# Autodesk Inventor assembly: Carrier
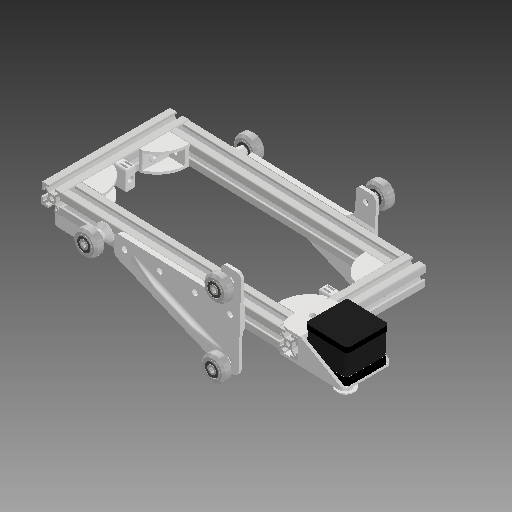
[picture p0: Inventor's stored thumbnail of the model, 512x512]
Saved by Autodesk Inventor 2020 (Build 240168000, 168)
## iProperties
Created: 2020-10-19
Part Number: Carrier
Document SubType Name: Assembly
Designer: DDeGo
Author: DDeGo
## Documents named in this file (13)
- C:\Users\DDeGo\Documents\Drew\Projects\De-Cruster\cad\Carrier.iam
- C:\Users\DDeGo\Documents\Drew\Projects\De-Cruster\cad\Cart Carrier.ipt
- C:\Users\DDeGo\Documents\Drew\Projects\De-Cruster\cad\VWheel.iam
- C:\Users\DDeGo\Documents\Drew\Projects\De-Cruster\cad\2020 Extrusion 200mm.ipt
- C:\Users\DDeGo\Documents\Drew\Projects\De-Cruster\cad\2020 Extrusion 122mm.ipt
- C:\Users\DDeGo\Documents\Drew\Projects\De-Cruster\cad\Nema 17.ipt
- C:\Users\DDeGo\Documents\Drew\Projects\De-Cruster\cad\GT2 Idler Pulley.ipt
- C:\Users\DDeGo\Documents\Drew\Projects\De-Cruster\cad\MotorBracket1.ipt
- C:\Users\DDeGo\Documents\Drew\Projects\De-Cruster\cad\ZBeltBlock.ipt
- C:\Users\DDeGo\Documents\Drew\Projects\De-Cruster\cad\HBLFSNF5_b.ipt
- C:\Users\DDeGo\Documents\Drew\Projects\De-Cruster\cad\YIdler.ipt
- C:\Users\DDeGo\Documents\Drew\Projects\De-Cruster\cad\SingleWheelPost.ipt
- C:\Users\DDeGo\Documents\Drew\Projects\De-Cruster\cad\Cart Carrier Mirrored.ipt
## Components (25 placed, 12 different names)
1. Cart Carrier:1 — Mate:1, Mate:2, Mate:12, Flush:5, Mate:17, Flush:26, Mate:46
2. VWheel:1 [sub-assembly] — Mate:1, Flush:1, Flush:2
3. VWheel:2 [sub-assembly] — Flush:2, Mate:43
4. VWheel:3 [sub-assembly] — Mate:2, Flush:1, Mate:12
5. VWheel:4 [sub-assembly] — Flush:3, Flush:4, Mate:49
6. VWheel:5 [sub-assembly] — Flush:4, Mate:42, Mate:47
7. VWheel:6 [sub-assembly] — Flush:3, Mate:48
8. 2020 Extrusion 200mm:1 — Flush:5, Flush:7, Flush:8, Flush:9, Flush:10, Flush:11, Mate:16, Mate:33, Mate:36, Flush:20, Mate:41, Mate:46
9. 2020 Extrusion 200mm:2 — Flush:7, Mate:15, Flush:13, Mate:28, Mate:34, Mate:35, Flush:19, Flush:21, Mate:40, Mate:44, Mate:45, Flush:25
10. 2020 Extrusion 122mm:1 — Mate:15, Flush:8, Flush:9, Mate:26, Flush:16, Mate:29, Mate:30, Flush:18, Mate:37, Flush:22, Flush:23
11. 2020 Extrusion 122mm:2 — Flush:10, Flush:11, Mate:16, Mate:17, Flush:13, Mate:21, Mate:22, Flush:14, Mate:27, Flush:15, Mate:31, Mate:32, Flush:24
12. Nema 17:1 — Mate:19, Mate:20, Mate:23, Mate:24, Mate:25
13. GT2 Idler Pulley:1 — Mate:19, Mate:20
14. GT2 Idler Pulley:2 — Mate:38, Mate:39
15. MotorBracket1:1 — Mate:21, Mate:22, Flush:14, Mate:23, Mate:24, Mate:25
16. ZBeltBlock:1 — Mate:26, Flush:16, Mate:28, Flush:17
17. ZBeltBlock:2 — Mate:27, Flush:15, Flush:17
18. HBLFSNF5_b:1 — Mate:29, Mate:36, Flush:18
19. HBLFSNF5_b:2 — Mate:30, Mate:35, Flush:19
20. HBLFSNF5_b:3 — Mate:31, Mate:33, Flush:20
21. HBLFSNF5_b:4 — Mate:32, Mate:34, Flush:21, Flush:24
22. YIdler:1 — Mate:37, Flush:22, Flush:23, Mate:38, Mate:39
23. SingleWheelPost:1 — Mate:40, Mate:42, Mate:47
24. SingleWheelPost:2 — Mate:41, Mate:43
25. Cart Carrier Mirrored:1 — Mate:44, Mate:45, Flush:25, Flush:26, Mate:48, Mate:49
## Relationships (61: Mate 37, Flush 24)
- Mate:1: Cart Carrier:1 ↔ VWheel:1
- Mate:2: Cart Carrier:1 ↔ VWheel:3
- Flush:1: VWheel:1 ↔ VWheel:3
- Flush:2: VWheel:1 ↔ VWheel:2
- Flush:3: VWheel:4 ↔ VWheel:6
- Flush:4: VWheel:4 ↔ VWheel:5
- Mate:12 (6 mm): Cart Carrier:1 ↔ VWheel:3
- Flush:5: Cart Carrier:1 ↔ 2020 Extrusion 200mm:1
- Flush:7: 2020 Extrusion 200mm:1 ↔ 2020 Extrusion 200mm:2
- Mate:15: 2020 Extrusion 200mm:2 ↔ 2020 Extrusion 122mm:1
- Flush:8: 2020 Extrusion 200mm:1 ↔ 2020 Extrusion 122mm:1
- Flush:9: 2020 Extrusion 200mm:1 ↔ 2020 Extrusion 122mm:1
- Flush:10: 2020 Extrusion 200mm:1 ↔ 2020 Extrusion 122mm:2
- Flush:11: 2020 Extrusion 200mm:1 ↔ 2020 Extrusion 122mm:2
- Mate:16: 2020 Extrusion 200mm:1 ↔ 2020 Extrusion 122mm:2
- Mate:17 (32.5 mm): Cart Carrier:1 ↔ 2020 Extrusion 122mm:2
- Flush:13: 2020 Extrusion 200mm:2 ↔ 2020 Extrusion 122mm:2
- Mate:19: Nema 17:1 ↔ GT2 Idler Pulley:1
- Mate:20 (10 mm): Nema 17:1 ↔ GT2 Idler Pulley:1
- Mate:21: 2020 Extrusion 122mm:2 ↔ MotorBracket1:1
- Mate:22: 2020 Extrusion 122mm:2 ↔ MotorBracket1:1
- Flush:14: 2020 Extrusion 122mm:2 ↔ MotorBracket1:1
- Mate:23: Nema 17:1 ↔ MotorBracket1:1
- Mate:24: Nema 17:1 ↔ MotorBracket1:1
- Mate:25: Nema 17:1 ↔ MotorBracket1:1
- Mate:26: 2020 Extrusion 122mm:1 ↔ ZBeltBlock:1
- Mate:27: 2020 Extrusion 122mm:2 ↔ ZBeltBlock:2
- Flush:15: 2020 Extrusion 122mm:2 ↔ ZBeltBlock:2
- Flush:16: 2020 Extrusion 122mm:1 ↔ ZBeltBlock:1
- Mate:28 (45 mm): 2020 Extrusion 200mm:2 ↔ ZBeltBlock:1
- Flush:17: ZBeltBlock:1 ↔ ZBeltBlock:2
- Mate:29: 2020 Extrusion 122mm:1 ↔ HBLFSNF5_b:1
- Mate:30: 2020 Extrusion 122mm:1 ↔ HBLFSNF5_b:2
- Mate:31: 2020 Extrusion 122mm:2 ↔ HBLFSNF5_b:3
- Mate:32: 2020 Extrusion 122mm:2 ↔ HBLFSNF5_b:4
- Mate:33: 2020 Extrusion 200mm:1 ↔ HBLFSNF5_b:3
- Mate:34: 2020 Extrusion 200mm:2 ↔ HBLFSNF5_b:4
- Mate:35: 2020 Extrusion 200mm:2 ↔ HBLFSNF5_b:2
- Mate:36: 2020 Extrusion 200mm:1 ↔ HBLFSNF5_b:1
- Flush:18: 2020 Extrusion 122mm:1 ↔ HBLFSNF5_b:1
- Flush:19: 2020 Extrusion 200mm:2 ↔ HBLFSNF5_b:2
- Flush:20: 2020 Extrusion 200mm:1 ↔ HBLFSNF5_b:3
- Flush:21: 2020 Extrusion 200mm:2 ↔ HBLFSNF5_b:4
- Mate:37: 2020 Extrusion 122mm:1 ↔ YIdler:1
- Flush:22: 2020 Extrusion 122mm:1 ↔ YIdler:1
- Flush:23 (-12 mm): 2020 Extrusion 122mm:1 ↔ YIdler:1
- Mate:38: GT2 Idler Pulley:2 ↔ YIdler:1
- Mate:39 (1 mm): GT2 Idler Pulley:2 ↔ YIdler:1
- Mate:40: 2020 Extrusion 200mm:2 ↔ SingleWheelPost:1
- Mate:41: 2020 Extrusion 200mm:1 ↔ SingleWheelPost:2
- Mate:42: VWheel:5 ↔ SingleWheelPost:1
- Mate:43: VWheel:2 ↔ SingleWheelPost:2
- Mate:44: 2020 Extrusion 200mm:2 ↔ Cart Carrier Mirrored:1
- Flush:24: 2020 Extrusion 122mm:2 ↔ HBLFSNF5_b:4
- Mate:45: 2020 Extrusion 200mm:2 ↔ Cart Carrier Mirrored:1
- Flush:25: 2020 Extrusion 200mm:2 ↔ Cart Carrier Mirrored:1
- Flush:26: Cart Carrier:1 ↔ Cart Carrier Mirrored:1
- Mate:46: Cart Carrier:1 ↔ 2020 Extrusion 200mm:1
- Mate:47: VWheel:5 ↔ SingleWheelPost:1
- Mate:48: VWheel:6 ↔ Cart Carrier Mirrored:1
- Mate:49: VWheel:4 ↔ Cart Carrier Mirrored:1
